# Autodesk Inventor assembly: FieldFinalTwo
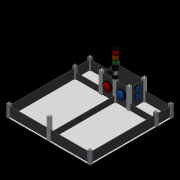
[picture p0: Inventor's stored thumbnail of the model, 180x180]
Saved by Autodesk Inventor 2016 (Build 200138000, 138)
## iProperties
Created: 2017-01-21
Part Number: FieldFinalTwo
Document SubType Name: Assembly
Designer: Alexis Renderos
Author: Alexis Renderos
## Documents named in this file (18)
- F:\Lego Robotics Missions\FieldFinalTwo.iam
- F:\Lego Robotics Missions\PolyBase.ipt
- F:\Lego Robotics Missions\ProfileTwo.ipt
- F:\Lego Robotics Missions\ProfileOne.ipt
- F:\Lego Robotics Missions\NLNMNMNR.ipt
- F:\Lego Robotics Missions\NLMFLNRMFR.ipt
- F:\Lego Robotics Missions\MFLSLMFRSR.ipt
- F:\Lego Robotics Missions\SLSMLSMRSR.ipt
- F:\Lego Robotics Missions\MFLMLMRMFR.ipt
- F:\Lego Robotics Missions\MLMRSMLSMR.ipt
- F:\Lego Robotics Missions\MLSMLMRSMR.ipt
- F:\Lego Robotics Missions\ButtonLargeBlue.ipt
- F:\Lego Robotics Missions\TowerLight.ipt
- F:\Lego Robotics Missions\NMMCMARK2.ipt
- F:\Lego Robotics Missions\MLMCMR.ipt
- F:\Lego Robotics Missions\ButtonLargeRed.ipt
- F:\Lego Robotics Missions\ButtonExtraLargeBlue.ipt
- F:\Lego Robotics Missions\ButtonExtraLargeRed.ipt
## Components (36 placed, 35 different names)
1. PolyBase:1 — Mate:1, Mate:2, Mate:3, Mate:4, Mate:5, Mate:6, Flush:1, Flush:2, Flush:3, Flush:4, Mate:7, Flush:5, Flush:6, Flush:7, Flush:8, Flush:9, Flush:10, Flush:11, Mate:8, Mate:9, Mate:10, Mate:11, Mate:12, Flush:12, Flush:13, Mate:16, Mate:17, Mate:20, Mate:22, Mate:26, Mate:28, Mate:30, Mate:32, Mate:34, Mate:35, Mate:40, Mate:42, Mate:44, Mate:56, Mate:59, Mate:60, Tangent:7, Tangent:8
2. NorthLeft — Mate:1, Flush:1, Flush:2, Symmetry:1, Mate:21, Flush:32
3. NorthMiddle — Mate:7, Flush:5, Mate:18, Mate:19, Mate:57
4. NorthRight — Mate:2, Flush:3, Flush:4, Symmetry:1, Mate:23, Flush:33, Flush:34
5. MiddleFarLeft — Mate:3, Flush:11, Flush:17, Mate:27, Mate:37, Flush:31
6. MiddleLeft — Mate:10, Flush:15, Flush:16, Flush:17, Symmetry:2, Mate:43, Flush:27, Symmetry:5, Symmetry:6, Mate:55, Symmetry:10
7. MiddleCenter — Mate:12, Mate:52, Mate:53, Mate:54, Mate:55, Mate:58, Mate:61, Mate:62, Mate:63, Symmetry:9, Symmetry:10
8. MiddleRight — Mate:11, Flush:14, Flush:16, Flush:18, Symmetry:2, Mate:45, Flush:23, Symmetry:7, Symmetry:8, Symmetry:9
9. MiddleFarRight — Mate:4, Flush:10, Flush:18, Mate:15, Mate:29, Mate:36, Flush:22
10. SouthLeft — Mate:5, Flush:6, Flush:7, Mate:13, Mate:31, Flush:28, Flush:29
11. SouthMiddleLeft — Mate:8, Flush:12, Flush:15, Mate:13, Flush:24, Flush:25, Symmetry:5, Symmetry:6
12. SouthMiddleRight — Mate:9, Flush:13, Flush:14, Mate:14, Mate:41, Symmetry:7, Symmetry:8
13. SouthRight — Mate:6, Flush:8, Flush:9, Mate:14, Mate:15, Mate:33, Flush:20, Flush:21
14. NL-MFL — Mate:20, Mate:21, Flush:31
15. NR-MFR — Mate:22, Mate:23, Flush:34
16. MFL-SL — Mate:26, Mate:27, Flush:29
17. ML-SML — Mate:42, Mate:43, Flush:25, Mate:48, Mate:49
18. MR-SMR — Mate:44, Mate:45, Flush:23, Mate:50, Mate:51
19. MFR-SR — Mate:28, Mate:29, Flush:20
20. NL-NM — Mate:16, Mate:19, Flush:32
21. NM-NR — Mate:17, Mate:18, Flush:33
22. MFL-ML — Mate:34, Mate:37, Flush:27, Tangent:3
23. MLMCMR:1 — Mate:59, Mate:61, Mate:63, Mate:64, Mate:65
24. MLMCMR:2 — Mate:60, Mate:62, Mate:64, Mate:66
25. MR-MFR — Mate:35, Mate:36, Flush:22, Tangent:5
26. SL-SML — Mate:30, Mate:31, Flush:28
27. SML-SMR — Mate:40, Mate:41, Flush:24
28. SMR-SR — Mate:32, Mate:33, Flush:21
29. RedTopButton — Mate:51, Tangent:6
30. RedBottomButton — Mate:50, Tangent:5, Tangent:6
31. BlueTopButton — Mate:49, Tangent:4
32. BlueBottomButton — Mate:48, Tangent:3, Tangent:4
33. NMMCMARK2:1 — Mate:56, Mate:57, Mate:58
34. TowerLight:1 — Mate:52, Mate:53, Mate:54
35. ButtonExtraLargeBlue:1 — Mate:65, Tangent:7
36. ButtonExtraLargeRed:1 — Mate:66, Tangent:8
## Relationships (105: Mate 60, Flush 31, Symmetry 8, Tangent 6)
- Mate:1: PolyBase:1 ↔ NorthLeft
- Mate:2: PolyBase:1 ↔ NorthRight
- Mate:3: PolyBase:1 ↔ MiddleFarLeft
- Mate:4: PolyBase:1 ↔ MiddleFarRight
- Mate:5: PolyBase:1 ↔ SouthLeft
- Mate:6: PolyBase:1 ↔ SouthRight
- Flush:1: PolyBase:1 ↔ NorthLeft
- Flush:2: PolyBase:1 ↔ NorthLeft
- Flush:3: PolyBase:1 ↔ NorthRight
- Flush:4: PolyBase:1 ↔ NorthRight
- Mate:7: PolyBase:1 ↔ NorthMiddle
- Flush:5: PolyBase:1 ↔ NorthMiddle
- Symmetry:1: NorthLeft ↔ NorthRight
- Flush:6: PolyBase:1 ↔ SouthLeft
- Flush:7: PolyBase:1 ↔ SouthLeft
- Flush:8: PolyBase:1 ↔ SouthRight
- Flush:9: PolyBase:1 ↔ SouthRight
- Flush:10: PolyBase:1 ↔ MiddleFarRight
- Flush:11: PolyBase:1 ↔ MiddleFarLeft
- Mate:8: PolyBase:1 ↔ SouthMiddleLeft
- Mate:9: PolyBase:1 ↔ SouthMiddleRight
- Mate:10: PolyBase:1 ↔ MiddleLeft
- Mate:11: PolyBase:1 ↔ MiddleRight
- Mate:12: PolyBase:1 ↔ MiddleCenter
- Flush:12: PolyBase:1 ↔ SouthMiddleLeft
- Flush:13: PolyBase:1 ↔ SouthMiddleRight
- Flush:14: MiddleRight ↔ SouthMiddleRight
- Flush:15: MiddleLeft ↔ SouthMiddleLeft
- Flush:16: MiddleLeft ↔ MiddleRight
- Mate:13 (279.4 mm): SouthLeft ↔ SouthMiddleLeft
- Mate:14 (279.4 mm): SouthMiddleRight ↔ SouthRight
- Flush:17: MiddleFarLeft ↔ MiddleLeft
- Flush:18: MiddleRight ↔ MiddleFarRight
- Symmetry:2: MiddleLeft ↔ MiddleRight
- Mate:15 (152.4 mm): MiddleFarRight ↔ SouthRight
- Mate:16: PolyBase:1 ↔ NL-NM
- Mate:17: PolyBase:1 ↔ NM-NR
- Mate:18: NorthMiddle ↔ NM-NR
- Mate:19: NorthMiddle ↔ NL-NM
- Mate:20: PolyBase:1 ↔ NL-MFL
- Mate:21: NorthLeft ↔ NL-MFL
- Mate:22: PolyBase:1 ↔ NR-MFR
- Mate:23: NorthRight ↔ NR-MFR
- Mate:26: PolyBase:1 ↔ MFL-SL
- Mate:27: MiddleFarLeft ↔ MFL-SL
- Mate:28: PolyBase:1 ↔ MFR-SR
- Mate:29: MiddleFarRight ↔ MFR-SR
- Mate:30: PolyBase:1 ↔ SL-SML
- Mate:31: SouthLeft ↔ SL-SML
- Mate:32: PolyBase:1 ↔ SMR-SR
- Mate:33: SouthRight ↔ SMR-SR
- Mate:34: PolyBase:1 ↔ MFL-ML
- Mate:35: PolyBase:1 ↔ MR-MFR
- Mate:36: MiddleFarRight ↔ MR-MFR
- Mate:37: MiddleFarLeft ↔ MFL-ML
- Mate:40: PolyBase:1 ↔ SML-SMR
- Mate:41: SouthMiddleRight ↔ SML-SMR
- Mate:42: PolyBase:1 ↔ ML-SML
- Mate:43: MiddleLeft ↔ ML-SML
- Mate:44: PolyBase:1 ↔ MR-SMR
- Mate:45: MiddleRight ↔ MR-SMR
- Flush:20: SouthRight ↔ MFR-SR
- Flush:21: SouthRight ↔ SMR-SR
- Flush:22: MiddleFarRight ↔ MR-MFR
- Flush:23: MiddleRight ↔ MR-SMR
- Flush:24: SouthMiddleLeft ↔ SML-SMR
- Flush:25: SouthMiddleLeft ↔ ML-SML
- Flush:27: MiddleLeft ↔ MFL-ML
- Flush:28: SouthLeft ↔ SL-SML
- Flush:29: SouthLeft ↔ MFL-SL
- Flush:31: MiddleFarLeft ↔ NL-MFL
- Flush:32: NorthLeft ↔ NL-NM
- Flush:33: NorthRight ↔ NM-NR
- Flush:34: NorthRight ↔ NR-MFR
- Mate:48: ML-SML ↔ BlueBottomButton
- Mate:49: ML-SML ↔ BlueTopButton
- Tangent:3: MFL-ML ↔ BlueBottomButton
- Symmetry:5: MiddleLeft ↔ SouthMiddleLeft
- Symmetry:6: MiddleLeft ↔ SouthMiddleLeft
- Tangent:4 (12.7 mm): BlueTopButton ↔ BlueBottomButton
- Mate:50: MR-SMR ↔ RedBottomButton
- Mate:51: MR-SMR ↔ RedTopButton
- Tangent:5: MR-MFR ↔ RedBottomButton
- Tangent:6 (12.7 mm): RedTopButton ↔ RedBottomButton
- Symmetry:7: MiddleRight ↔ SouthMiddleRight
- Symmetry:8: MiddleRight ↔ SouthMiddleRight
- Mate:52: MiddleCenter ↔ TowerLight:1
- Mate:53: MiddleCenter ↔ TowerLight:1
- Mate:54: MiddleCenter ↔ TowerLight:1
- Mate:55: MiddleLeft ↔ MiddleCenter
- Mate:56: PolyBase:1 ↔ NMMCMARK2:1
- Mate:57: NorthMiddle ↔ NMMCMARK2:1
- Mate:58: MiddleCenter ↔ NMMCMARK2:1
- Mate:59: PolyBase:1 ↔ MLMCMR:1
- Mate:60: PolyBase:1 ↔ MLMCMR:2
- Mate:61: MiddleCenter ↔ MLMCMR:1
- Mate:62: MiddleCenter ↔ MLMCMR:2
- Mate:63: MiddleCenter ↔ MLMCMR:1
- Mate:64: MLMCMR:1 ↔ MLMCMR:2
- Mate:65: MLMCMR:1 ↔ ButtonExtraLargeBlue:1
- Mate:66: MLMCMR:2 ↔ ButtonExtraLargeRed:1
- Symmetry:9: MiddleCenter ↔ MiddleRight
- Symmetry:10: MiddleLeft ↔ MiddleCenter
- Tangent:7 (63.5 mm): PolyBase:1 ↔ ButtonExtraLargeBlue:1
- Tangent:8 (63.5 mm): PolyBase:1 ↔ ButtonExtraLargeRed:1
